# Autodesk Inventor assembly: PaddleCollection2.1.ipt
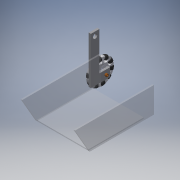
[picture p0: Inventor's stored thumbnail of the model, 180x180]
Saved by Autodesk Inventor 2019 (Build 230136000, 136)
## iProperties
Created: 2018-10-20
Part Number: PaddleCollection2.1.ipt
Document SubType Name: Assembly
Designer: User
Author: User
## Documents named in this file (8)
- C:\Robotics\CAD\2018-19_CAD\Collection\PaddleCollection2.1.ipt.iam
- C:\Robotics\CAD\2018-19_CAD\Collection\PaddleCollection2.1AxleSupport.ipt
- C:\Robotics\CAD\2018-19_CAD\Collection\PaddleCollection2.1Casing.ipt
- C:\Robotics\CAD\2018-19_CAD\Collection\PaddleCollectionFloor.ipt
- C:\Robotics\CAD\COTSParts\Tetrix\Tetrix Wheel 3 in omni.ipt
- C:\Robotics\CAD\COTSParts\Tetrix\Bronze bushing.ipt
- C:\Robotics\CAD\COTSParts\Tetrix\Tetrix shaft collar.ipt
- C:\Robotics\CAD\COTSParts\Tetrix\Tetrix Hub - axle.ipt
## Components (9 placed, 7 different names)
1. PaddleCollection2.1AxleSupport:1 — Mate:1, Mate:2, Flush:1, Insert:1
2. PaddleCollection2.1Casing:1 — Flush:3, Mate:5, Mate:6, Mate:1
3. PaddleCollection2.1Casing:2 — Mate:3, Mate:4, Flush:2
4. PaddleCollectionFloor:1 — Mate:2, Flush:1, Mate:3, Mate:4, Flush:2, Flush:3, Mate:5, Mate:6
5. Tetrix Wheel 3 in omni:1 — Insert:3, Insert:4
6. Bronze bushing:1 — Insert:1, Insert:2
7. Bronze bushing:2 — Insert:5
8. Tetrix shaft collar:1 — Insert:2, Insert:3
9. Tetrix Hub - axle:1 — Insert:4, Insert:5
## Relationships (14: Mate 6, Insert 5, Flush 3)
- Mate:1: PaddleCollection2.1AxleSupport:1 ↔ PaddleCollection2.1Casing:1
- Mate:2: PaddleCollection2.1AxleSupport:1 ↔ PaddleCollectionFloor:1
- Flush:1: PaddleCollection2.1AxleSupport:1 ↔ PaddleCollectionFloor:1
- Mate:3: PaddleCollection2.1Casing:2 ↔ PaddleCollectionFloor:1
- Mate:4: PaddleCollection2.1Casing:2 ↔ PaddleCollectionFloor:1
- Flush:2: PaddleCollection2.1Casing:2 ↔ PaddleCollectionFloor:1
- Flush:3: PaddleCollection2.1Casing:1 ↔ PaddleCollectionFloor:1
- Mate:5: PaddleCollection2.1Casing:1 ↔ PaddleCollectionFloor:1
- Mate:6: PaddleCollection2.1Casing:1 ↔ PaddleCollectionFloor:1
- Insert:1: PaddleCollection2.1AxleSupport:1 ↔ Bronze bushing:1
- Insert:2: Bronze bushing:1 ↔ Tetrix shaft collar:1
- Insert:3: Tetrix Wheel 3 in omni:1 ↔ Tetrix shaft collar:1
- Insert:4: Tetrix Wheel 3 in omni:1 ↔ Tetrix Hub - axle:1
- Insert:5: Bronze bushing:2 ↔ Tetrix Hub - axle:1
